# Autodesk Inventor assembly: NEMA 17 Stepper Motor Assembly
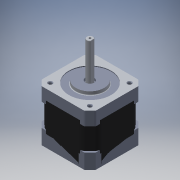
[picture p0: Inventor's stored thumbnail of the model, 180x180]
Saved by Autodesk Inventor 2016 (Build 200138000, 138)
## iProperties
Created: 2013-05-26
Part Number: NEMA 17 Stepper Motor Assembly
Document SubType Name: Assembly
Designer: Scott
Sending System: SolidWorks 2012
Last Author: Brian
Last Saved: 2013-05-26
Author: Scott
## Documents named in this file (6)
- E:\Scott Projects\3D Printing\CoreXY\NEMA 17 Stepper Motor Assembly.iam
- E:\Scott Projects\3D Printing\CoreXY\Downloaded parts\nema-17-stepper-motor-1.snapshot.2\NEMA 17 Stepper Motor Middle.ipt
- E:\Scott Projects\3D Printing\CoreXY\Downloaded parts\nema-17-stepper-motor-1.snapshot.2\NEMA 17 Stepper Motor Top.ipt
- E:\Scott Projects\3D Printing\CoreXY\Downloaded parts\nema-17-stepper-motor-1.snapshot.2\NEMA 17 Stepper Motor Bottom.ipt
- E:\Scott Projects\3D Printing\CoreXY\Downloaded parts\nema-17-stepper-motor-1.snapshot.2\NEMA 17 Stepper Motor Shaft.ipt
- E:\Scott Projects\3D Printing\CoreXY\Downloaded parts\nema-17-stepper-motor-1.snapshot.2\pan cross head_am.ipt
## Components (8 placed, 5 different names)
1. NEMA 17 Stepper Motor Middle:1 — Flush:1, Mate:2, Mate:3
2. NEMA 17 Stepper Motor Top:1 — Mate:1, Flush:2, Flush:3, Mate:3
3. NEMA 17 Stepper Motor Bottom:1 — Mate:1, Flush:1, Flush:2, Flush:3, Mate:2, Insert:1, Insert:2, Insert:3, Insert:4, Insert:5
4. NEMA 17 Stepper Motor Shaft:1 — Insert:5
5. pan cross head_am:1 — Insert:1
6. pan cross head_am:2 — Insert:4
7. pan cross head_am:3 — Insert:3
8. pan cross head_am:4 — Insert:2
## Relationships (11: Insert 5, Mate 3, Flush 3)
- Mate:1 (-40 mm): NEMA 17 Stepper Motor Top:1 ↔ NEMA 17 Stepper Motor Bottom:1
- Flush:1: NEMA 17 Stepper Motor Middle:1 ↔ NEMA 17 Stepper Motor Bottom:1
- Flush:2: NEMA 17 Stepper Motor Top:1 ↔ NEMA 17 Stepper Motor Bottom:1
- Flush:3: NEMA 17 Stepper Motor Top:1 ↔ NEMA 17 Stepper Motor Bottom:1
- Mate:2: NEMA 17 Stepper Motor Middle:1 ↔ NEMA 17 Stepper Motor Bottom:1
- Mate:3: NEMA 17 Stepper Motor Middle:1 ↔ NEMA 17 Stepper Motor Top:1
- Insert:1: NEMA 17 Stepper Motor Bottom:1 ↔ pan cross head_am:1
- Insert:2: NEMA 17 Stepper Motor Bottom:1 ↔ pan cross head_am:4
- Insert:3: NEMA 17 Stepper Motor Bottom:1 ↔ pan cross head_am:3
- Insert:4: NEMA 17 Stepper Motor Bottom:1 ↔ pan cross head_am:2
- Insert:5: NEMA 17 Stepper Motor Bottom:1 ↔ NEMA 17 Stepper Motor Shaft:1
